# Autodesk Inventor assembly: Upper Stage
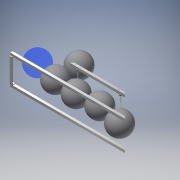
[picture p0: Inventor's stored thumbnail of the model, 180x180]
Saved by Autodesk Inventor 2019.4 (Build 234330000, 330)
## iProperties
Created: 2020-01-18
Part Number: Upper Stage
Document SubType Name: Assembly
Designer: Mark
Mass: 1292.77 g
Surface Area: 4691.82 cm^2
Volume: 478.802 cm^3
Density: 2.7 g/cm^3
Author: Mark
## Documents named in this file (8)
- C:\Users\Mark\Desktop\7738 Helion Engineering\7738-2020\Upper Stage\Upper Stage.iam
- C:\Users\Mark\Desktop\7738 Helion Engineering\7738-2020\Upper Stage\Main Extrusions.ipt
- C:\Users\Mark\Desktop\7738 Helion Engineering\7738-2020\Upper Stage\Back Support Piece.ipt
- C:\Users\Mark\Desktop\7738 Helion Engineering\7738-2020\Upper Stage\Secondary Extrusions.ipt
- C:\Users\Mark\Desktop\7738 Helion Engineering\7738-2020\Power Cell.ipt
- C:\Users\Mark\Desktop\7738 Helion Engineering\7738-2020\Upper Stage\First stage shaft.ipt
- C:\Users\Mark\Desktop\7738 Helion Engineering\7738-2020\Upper Stage\KFL08.ipt
- C:\Users\Mark\Desktop\7738 Helion Engineering\7738-2020\Upper Stage\Turret Support.ipt
## Components (16 placed, 7 different names)
1. Main Extrusions:1 — Mate:1, Flush:1, Flush:2, Flush:8, Flush:11, Mate:20, Mate:21
2. Main Extrusions:2 — Mate:1, Flush:1, Flush:2, Flush:3, Flush:4, Mate:2, Flush:5, Flush:7, Mate:3
3. Back Support Piece:1 — Flush:3, Flush:4, Mate:2
4. Secondary Extrusions:1 — Flush:5, Flush:7, Flush:9, Mate:3, Flush:10, Mate:4, Mate:5, Mate:6, Mate:13, Mate:14, Mate:15
5. Secondary Extrusions:2 — Flush:8, Flush:9, Flush:10, Mate:7, Mate:8, Mate:9, Mate:10, Mate:11, Mate:12
6. Power Cell:1
7. Power Cell:2
8. Power Cell:3
9. Power Cell:4
10. First stage shaft:1 — Mate:16, Mate:17
11. KFL08:1 — Mate:4, Mate:5, Mate:6
12. KFL08:2 — Mate:7, Mate:8, Mate:9, Mate:16, Mate:17
13. KFL08:3 — Mate:13, Mate:14, Mate:15
14. KFL08:4 — Mate:10, Mate:11, Mate:12, Mate:18, Mate:19
15. First stage shaft:2 — Mate:18, Mate:19
16. Turret Support:1 — Flush:11, Mate:20, Mate:21
## Relationships (31: Mate 21, Flush 10)
- Mate:1 (200 mm): Main Extrusions:1 ↔ Main Extrusions:2
- Flush:1: Main Extrusions:1 ↔ Main Extrusions:2
- Flush:2: Main Extrusions:1 ↔ Main Extrusions:2
- Flush:3: Main Extrusions:2 ↔ Back Support Piece:1
- Flush:4: Main Extrusions:2 ↔ Back Support Piece:1
- Mate:2: Main Extrusions:2 ↔ Back Support Piece:1
- Flush:5: Main Extrusions:2 ↔ Secondary Extrusions:1
- Flush:7: Main Extrusions:2 ↔ Secondary Extrusions:1
- Flush:8: Main Extrusions:1 ↔ Secondary Extrusions:2
- Flush:9: Secondary Extrusions:1 ↔ Secondary Extrusions:2
- Mate:3 (150 mm): Main Extrusions:2 ↔ Secondary Extrusions:1
- Flush:10: Secondary Extrusions:1 ↔ Secondary Extrusions:2
- Mate:4: Secondary Extrusions:1 ↔ KFL08:1
- Mate:5: Secondary Extrusions:1 ↔ KFL08:1
- Mate:6: Secondary Extrusions:1 ↔ KFL08:1
- Mate:7: Secondary Extrusions:2 ↔ KFL08:2
- Mate:8: Secondary Extrusions:2 ↔ KFL08:2
- Mate:9: Secondary Extrusions:2 ↔ KFL08:2
- Mate:10: Secondary Extrusions:2 ↔ KFL08:4
- Mate:11: Secondary Extrusions:2 ↔ KFL08:4
- Mate:12: Secondary Extrusions:2 ↔ KFL08:4
- Mate:13: Secondary Extrusions:1 ↔ KFL08:3
- Mate:14: Secondary Extrusions:1 ↔ KFL08:3
- Mate:15: Secondary Extrusions:1 ↔ KFL08:3
- Mate:16: First stage shaft:1 ↔ KFL08:2
- Mate:17 (0.2 mm): First stage shaft:1 ↔ KFL08:2
- Mate:18: KFL08:4 ↔ First stage shaft:2
- Mate:19 (0.2 mm): KFL08:4 ↔ First stage shaft:2
- Flush:11: Main Extrusions:1 ↔ Turret Support:1
- Mate:20: Main Extrusions:1 ↔ Turret Support:1
- Mate:21: Main Extrusions:1 ↔ Turret Support:1
